# Autodesk Inventor assembly: Test slider
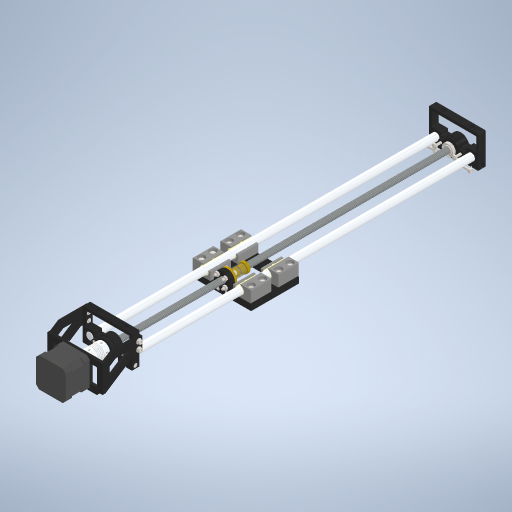
[picture p0: Inventor's stored thumbnail of the model, 512x512]
Saved by Autodesk Inventor 2023.2 (Build 272271000, 271)
## iProperties
Created: 2018-08-24
Part Number: Test slider
Description: STEP AP214
Document SubType Name: Assembly
Designer: Ayoub
Sending System: SolidWorks 2017
Preprocessor: SwSTEP 2.0
Title: Test slider.STEP
Revision Number: ANY
## Documents named in this file (23)
- C:\Users\Ayoub\Documents\GitHub\zonnepaneel-concept\Parts\Test slider\Test slider.iam
- C:\Users\Ayoub\Documents\GitHub\zonnepaneel-concept\Parts\Nema17 Stepper motor.ipt
- C:\Users\Ayoub\Documents\GitHub\zonnepaneel-concept\Parts\Flexible coupling D20 d5.ipt
- C:\Users\Ayoub\Documents\GitHub\zonnepaneel-concept\Parts\Trapezoidal lead screw tr8x8-4.ipt
- C:\Users\Ayoub\Documents\GitHub\zonnepaneel-concept\Parts\radial ball bearing_68_skf_SKF - 626 - 8,SI,NC,8_68.ipt
- C:\Users\Ayoub\Documents\GitHub\zonnepaneel-concept\Parts\hex thin nut chamfered gradeab_din_Hexagon Thin Nut ISO 4035 - M6 - N.ipt
- C:\Users\Ayoub\Documents\GitHub\zonnepaneel-concept\Parts\radial ball bearing_68_skf_SKF - 618-8 - 12,SI,NC,12_68.ipt
- C:\Users\Ayoub\Documents\GitHub\zonnepaneel-concept\Parts\d10 guide^Test slider.ipt
- C:\Users\Ayoub\Documents\GitHub\zonnepaneel-concept\Parts\T8 Antibacklash nut.iam
- C:\Users\Ayoub\Documents\GitHub\zonnepaneel-concept\Parts\WJ200UM_01_10_2.ipt
- C:\Users\Ayoub\Documents\GitHub\zonnepaneel-concept\Parts\Test slider support 1.ipt
- C:\Users\Ayoub\Documents\GitHub\zonnepaneel-concept\Parts\Test slider carriage small_double.ipt
- C:\Users\Ayoub\Documents\GitHub\zonnepaneel-concept\Parts\socket head cap screw_din_DIN 912 M6 x 16 --- 16N.ipt
- C:\Users\Ayoub\Documents\GitHub\zonnepaneel-concept\Parts\Test slider nut bracket.ipt
- C:\Users\Ayoub\Documents\GitHub\zonnepaneel-concept\Parts\socket head cap screw_din_DIN 912 M3 x 16 --- 16N.ipt
- C:\Users\Ayoub\Documents\GitHub\zonnepaneel-concept\Parts\hex nut style 1 gradeab_din_Hexagon Nut ISO 4032 - M3 - D - N.ipt
- C:\Users\Ayoub\Documents\GitHub\zonnepaneel-concept\Parts\socket head cap screw_din_DIN 912 M3 x 10 --- 10N.ipt
- C:\Users\Ayoub\Documents\GitHub\zonnepaneel-concept\Parts\Test slider support 1 cover.ipt
- C:\Users\Ayoub\Documents\GitHub\zonnepaneel-concept\Parts\socket head cap screw_din_DIN 912 M3 x 12 --- 12N.ipt
- C:\Users\Ayoub\Documents\GitHub\zonnepaneel-concept\Parts\Test slider support 2.ipt
- C:\Users\Ayoub\Documents\GitHub\zonnepaneel-concept\Parts\Test slider support 2 cover.ipt
- C:\Users\Ayoub\Documents\GitHub\zonnepaneel-concept\Parts\Test slider stepper mount.ipt
- C:\Users\Ayoub\Documents\GitHub\zonnepaneel-concept\Parts\plain washer grade a_din_Washer DIN 125 - A 3.2.ipt
## Components (76 placed, 76 different names)
1. Nema17 Stepper motor_1
2. Flexible coupling D20 d5_2
3. Trapezoidal lead screw tr8x8-4_3 — Mate:4
4. radial ball bearing_68_skf_SKF - 626 - 8,SI,NC,8_68_4
5. hex thin nut chamfered gradeab_din_Hexagon Thin Nut ISO 4035 - M6 - N_5
6. radial ball bearing_68_skf_SKF - 618-8 - 12,SI,NC,12_68_6
7. d10 guide^Test slider_7 — Insert:19
8. T8 Antibacklash nut_8 [sub-assembly] — Mate:2, Mate:3, Insert:1, Insert:2, Insert:3, Insert:4
9. WJ200UM_01_10_2_9 — Insert:17, Mate:20
10. d10 guide^Test slider_10 — Insert:18, Insert:26, Mate:20
11. Test slider support 1_11 — Insert:18
12. WJ200UM_01_10_2_12 — Insert:23, Insert:30
13. Test slider carriage small_double_13 — Mate:10, Mate:11, Insert:9, Insert:10, Insert:11, Insert:12, Insert:13, Insert:14, Insert:15, Insert:16
14. socket head cap screw_din_DIN 912 M6 x 16 --- 16N_14 — Insert:14, Insert:17
15. socket head cap screw_din_DIN 912 M6 x 16 --- 16N_15 — Insert:13
16. socket head cap screw_din_DIN 912 M6 x 16 --- 16N_16 — Insert:9, Insert:23
17. socket head cap screw_din_DIN 912 M6 x 16 --- 16N_17 — Insert:10, Insert:30
18. Test slider nut bracket_18 — Mate:2, Mate:3, Mate:4, Mate:6, Mate:7, Mate:8, Mate:9, Insert:5, Insert:6
19. socket head cap screw_din_DIN 912 M3 x 16 --- 16N_19 — Insert:4
20. socket head cap screw_din_DIN 912 M3 x 16 --- 16N_20 — Insert:3
21. socket head cap screw_din_DIN 912 M3 x 16 --- 16N_21 — Insert:1
22. socket head cap screw_din_DIN 912 M3 x 16 --- 16N_22 — Insert:2
23. hex nut style 1 gradeab_din_Hexagon Nut ISO 4032 - M3 - D - N_23 — Mate:7
24. hex nut style 1 gradeab_din_Hexagon Nut ISO 4032 - M3 - D - N_24 — Mate:9
25. hex nut style 1 gradeab_din_Hexagon Nut ISO 4032 - M3 - D - N_25 — Mate:6
26. hex nut style 1 gradeab_din_Hexagon Nut ISO 4032 - M3 - D - N_26 — Mate:8
27. socket head cap screw_din_DIN 912 M3 x 10 --- 10N_27 — Insert:6, Insert:7
28. socket head cap screw_din_DIN 912 M3 x 10 --- 10N_28 — Insert:5, Insert:8
29. hex nut style 1 gradeab_din_Hexagon Nut ISO 4032 - M3 - D - N_29
30. socket head cap screw_din_DIN 912 M3 x 16 --- 16N_30
31. socket head cap screw_din_DIN 912 M3 x 16 --- 16N_31
32. hex nut style 1 gradeab_din_Hexagon Nut ISO 4032 - M3 - D - N_32
33. Test slider support 1 cover_33
34. socket head cap screw_din_DIN 912 M3 x 12 --- 12N_34
35. socket head cap screw_din_DIN 912 M3 x 12 --- 12N_35
36. hex nut style 1 gradeab_din_Hexagon Nut ISO 4032 - M3 - D - N_36
37. hex nut style 1 gradeab_din_Hexagon Nut ISO 4032 - M3 - D - N_37
38. Test slider support 2_38 — Insert:19, Insert:20, Insert:26, Insert:27
39. Test slider support 2 cover_39
40. Test slider stepper mount_40 — Insert:20, Mate:18, Mate:19, Insert:27
41. plain washer grade a_din_Washer DIN 125 - A 3.2_41
42. plain washer grade a_din_Washer DIN 125 - A 3.2_42
43. plain washer grade a_din_Washer DIN 125 - A 3.2_43
44. plain washer grade a_din_Washer DIN 125 - A 3.2_44
45. socket head cap screw_din_DIN 912 M3 x 10 --- 10N_45
46. socket head cap screw_din_DIN 912 M3 x 10 --- 10N_46
47. socket head cap screw_din_DIN 912 M3 x 10 --- 10N_47
48. socket head cap screw_din_DIN 912 M3 x 10 --- 10N_48
49. plain washer grade a_din_Washer DIN 125 - A 3.2_49
50. plain washer grade a_din_Washer DIN 125 - A 3.2_50
51. socket head cap screw_din_DIN 912 M3 x 10 --- 10N_51
52. socket head cap screw_din_DIN 912 M3 x 10 --- 10N_52
53. hex nut style 1 gradeab_din_Hexagon Nut ISO 4032 - M3 - D - N_53
54. hex nut style 1 gradeab_din_Hexagon Nut ISO 4032 - M3 - D - N_54
55. hex nut style 1 gradeab_din_Hexagon Nut ISO 4032 - M3 - D - N_55
56. hex nut style 1 gradeab_din_Hexagon Nut ISO 4032 - M3 - D - N_56
57. hex nut style 1 gradeab_din_Hexagon Nut ISO 4032 - M3 - D - N_57
58. hex nut style 1 gradeab_din_Hexagon Nut ISO 4032 - M3 - D - N_58
59. socket head cap screw_din_DIN 912 M3 x 16 --- 16N_59
60. socket head cap screw_din_DIN 912 M3 x 16 --- 16N_60
61. socket head cap screw_din_DIN 912 M3 x 12 --- 12N_61
62. socket head cap screw_din_DIN 912 M3 x 12 --- 12N_62
63. plain washer grade a_din_Washer DIN 125 - A 3.2_63 — Mate:18, Insert:21
64. plain washer grade a_din_Washer DIN 125 - A 3.2_64 — Mate:19, Insert:22
65. socket head cap screw_din_DIN 912 M3 x 10 --- 10N_65 — Insert:21
66. socket head cap screw_din_DIN 912 M3 x 10 --- 10N_66 — Insert:22
67. hex nut style 1 gradeab_din_Hexagon Nut ISO 4032 - M3 - D - N_67
68. hex nut style 1 gradeab_din_Hexagon Nut ISO 4032 - M3 - D - N_68
69. socket head cap screw_din_DIN 912 M6 x 16 --- 16N_69 — Insert:16, Insert:28
70. socket head cap screw_din_DIN 912 M6 x 16 --- 16N_70 — Insert:15, Insert:24
71. socket head cap screw_din_DIN 912 M6 x 16 --- 16N_71 — Insert:11, Insert:29
72. socket head cap screw_din_DIN 912 M6 x 16 --- 16N_72 — Insert:12, Insert:25
73. WJ200UM_01_10_2_73 — Insert:25, Insert:29
74. WJ200UM_01_10_2_74 — Insert:24, Insert:28
75. hex nut style 1 gradeab_din_Hexagon Nut ISO 4032 - M3 - D - N_75 — Mate:10, Insert:7
76. hex nut style 1 gradeab_din_Hexagon Nut ISO 4032 - M3 - D - N_76 — Mate:11, Insert:8
## Relationships (42: Insert 30, Mate 12)
- Mate:2: T8 Antibacklash nut_8 ↔ Test slider nut bracket_18
- Mate:3: T8 Antibacklash nut_8 ↔ Test slider nut bracket_18
- Mate:4: Trapezoidal lead screw tr8x8-4_3 ↔ Test slider nut bracket_18
- Insert:1: T8 Antibacklash nut_8 ↔ socket head cap screw_din_DIN 912 M3 x 16 --- 16N_21
- Insert:2: T8 Antibacklash nut_8 ↔ socket head cap screw_din_DIN 912 M3 x 16 --- 16N_22
- Mate:6: Test slider nut bracket_18 ↔ hex nut style 1 gradeab_din_Hexagon Nut ISO 4032 - M3 - D - N_25
- Mate:7: Test slider nut bracket_18 ↔ hex nut style 1 gradeab_din_Hexagon Nut ISO 4032 - M3 - D - N_23
- Mate:8: Test slider nut bracket_18 ↔ hex nut style 1 gradeab_din_Hexagon Nut ISO 4032 - M3 - D - N_26
- Insert:3: T8 Antibacklash nut_8 ↔ socket head cap screw_din_DIN 912 M3 x 16 --- 16N_20
- Insert:4: T8 Antibacklash nut_8 ↔ socket head cap screw_din_DIN 912 M3 x 16 --- 16N_19
- Mate:9: Test slider nut bracket_18 ↔ hex nut style 1 gradeab_din_Hexagon Nut ISO 4032 - M3 - D - N_24
- Insert:5: Test slider nut bracket_18 ↔ socket head cap screw_din_DIN 912 M3 x 10 --- 10N_28
- Insert:6: Test slider nut bracket_18 ↔ socket head cap screw_din_DIN 912 M3 x 10 --- 10N_27
- Mate:10: Test slider carriage small_double_13 ↔ hex nut style 1 gradeab_din_Hexagon Nut ISO 4032 - M3 - D - N_75
- Mate:11: Test slider carriage small_double_13 ↔ hex nut style 1 gradeab_din_Hexagon Nut ISO 4032 - M3 - D - N_76
- Insert:7: socket head cap screw_din_DIN 912 M3 x 10 --- 10N_27 ↔ hex nut style 1 gradeab_din_Hexagon Nut ISO 4032 - M3 - D - N_75
- Insert:8: socket head cap screw_din_DIN 912 M3 x 10 --- 10N_28 ↔ hex nut style 1 gradeab_din_Hexagon Nut ISO 4032 - M3 - D - N_76
- Insert:9: Test slider carriage small_double_13 ↔ socket head cap screw_din_DIN 912 M6 x 16 --- 16N_16
- Insert:10: Test slider carriage small_double_13 ↔ socket head cap screw_din_DIN 912 M6 x 16 --- 16N_17
- Insert:11: Test slider carriage small_double_13 ↔ socket head cap screw_din_DIN 912 M6 x 16 --- 16N_71
- Insert:12: Test slider carriage small_double_13 ↔ socket head cap screw_din_DIN 912 M6 x 16 --- 16N_72
- Insert:13: Test slider carriage small_double_13 ↔ socket head cap screw_din_DIN 912 M6 x 16 --- 16N_15
- Insert:14: Test slider carriage small_double_13 ↔ socket head cap screw_din_DIN 912 M6 x 16 --- 16N_14
- Insert:15: Test slider carriage small_double_13 ↔ socket head cap screw_din_DIN 912 M6 x 16 --- 16N_70
- Insert:16: Test slider carriage small_double_13 ↔ socket head cap screw_din_DIN 912 M6 x 16 --- 16N_69
- Insert:17 (-2.5 mm): WJ200UM_01_10_2_9 ↔ socket head cap screw_din_DIN 912 M6 x 16 --- 16N_14
- Insert:18: d10 guide^Test slider_10 ↔ Test slider support 1_11
- Insert:19: d10 guide^Test slider_7 ↔ Test slider support 2_38
- Insert:20: Test slider support 2_38 ↔ Test slider stepper mount_40
- Mate:18: Test slider stepper mount_40 ↔ plain washer grade a_din_Washer DIN 125 - A 3.2_63
- Insert:21: plain washer grade a_din_Washer DIN 125 - A 3.2_63 ↔ socket head cap screw_din_DIN 912 M3 x 10 --- 10N_65
- Mate:19: Test slider stepper mount_40 ↔ plain washer grade a_din_Washer DIN 125 - A 3.2_64
- Insert:22: plain washer grade a_din_Washer DIN 125 - A 3.2_64 ↔ socket head cap screw_din_DIN 912 M3 x 10 --- 10N_66
- Insert:23: WJ200UM_01_10_2_12 ↔ socket head cap screw_din_DIN 912 M6 x 16 --- 16N_16
- Insert:24: socket head cap screw_din_DIN 912 M6 x 16 --- 16N_70 ↔ WJ200UM_01_10_2_74
- Insert:25: socket head cap screw_din_DIN 912 M6 x 16 --- 16N_72 ↔ WJ200UM_01_10_2_73
- Insert:26: d10 guide^Test slider_10 ↔ Test slider support 2_38
- Insert:27: Test slider support 2_38 ↔ Test slider stepper mount_40
- Insert:28: socket head cap screw_din_DIN 912 M6 x 16 --- 16N_69 ↔ WJ200UM_01_10_2_74
- Insert:29: socket head cap screw_din_DIN 912 M6 x 16 --- 16N_71 ↔ WJ200UM_01_10_2_73
- Insert:30: WJ200UM_01_10_2_12 ↔ socket head cap screw_din_DIN 912 M6 x 16 --- 16N_17
- Mate:20: WJ200UM_01_10_2_9 ↔ d10 guide^Test slider_10
